# Autodesk Inventor assembly: Robot Assembly V1.5 - 6 wheel - toughbox mini - 24x28
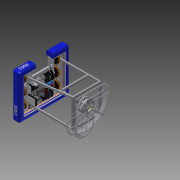
[picture p0: Inventor's stored thumbnail of the model, 180x180]
Saved by Autodesk Inventor 2013 (Build 170138000, 138)
## iProperties
Created: 2013-01-06
Part Number: Robot Assembly V1.5 - 6 wheel - toughbox mini - 24x28
Document SubType Name: Assembly
Designer: Moses
Mass: 19140.8 g
Surface Area: 65318.4 cm^2
Volume: 26385.5 cm^3
Density: 0.72543 g/cm^3
Author: Moses
## Documents named in this file (31)
- C:\Users\Moses\Documents\GitHub\frc2013CAD\Robot Assembly V1.5 - 6 wheel - toughbox mini - 24x28.iam
- C:\Users\Moses\Documents\GitHub\frc2013CAD\Drivetrain\Bearings\fr8zz-hex.ipt
- C:\Users\Moses\Documents\GitHub\frc2013CAD\Drivetrain\Drive Wheel Assembly V2.iam
- C:\Users\Moses\Documents\GitHub\frc2013CAD\Drivetrain\Standard Wheel Assembly V2.iam
- C:\Users\Moses\Documents\GitHub\frc2013CAD\Drivetrain\Toughbox-mini\Toughbox-mini-hex-long.iam
- C:\Users\Moses\Documents\GitHub\frc2013CAD\Drivetrain\6157K140 Shaft Collar\6157K140.ipt
- C:\Users\Moses\Documents\GitHub\frc2013CAD\Drivetrain\Shaft Spacer Part1.ipt
- C:\Users\Moses\Documents\GitHub\frc2013CAD\Drivetrain\Shaft Spacer Part2.ipt
- C:\Users\Moses\Documents\GitHub\frc2013CAD\Drivetrain\Shaft Spacer Part3.ipt
- C:\Users\Moses\Documents\GitHub\frc2013CAD\Drivetrain\Shaft Spacer Part4.ipt
- C:\Users\Moses\Documents\GitHub\frc2013CAD\Drivetrain\Shaft Spacer Part5.ipt
- C:\Users\Moses\Documents\GitHub\frc2013CAD\Drivetrain\Shaft Spacer Part6.ipt
- C:\Users\Moses\Documents\GitHub\frc2013CAD\Electrical\ELEC_Battery_NP18-12B.iam
- C:\Users\Moses\Documents\GitHub\frc2013CAD\Drivetrain\6061K130 Shaft\6061K130.ipt
- C:\Users\Moses\Documents\GitHub\frc2013CAD\Electrical\ELEC_CircuitBreaker_CB185-120.iam
- C:\Users\Moses\Documents\GitHub\frc2013CAD\Control Systems\CS_PowerBoard_A003206.ipt
- C:\Users\Moses\Documents\GitHub\frc2013CAD\Control Systems\CS_compactRIO_cRIO-FRC-II.ipt
- C:\Users\Moses\Documents\GitHub\frc2013CAD\Control Systems\CS_WirelessBridge_DAP1522.ipt
- C:\Users\Moses\Documents\GitHub\frc2013CAD\Control Systems\CS_Converter_CLL25-24S05.ipt
- C:\Users\Moses\Documents\GitHub\frc2013CAD\Control Systems\Talon.ipt
- C:\Users\Moses\Documents\GitHub\frc2013CAD\Drivetrain\Pneumatic_Compressor_VIAIR_00090\Pneumatic_Compressor_VIAIR_00090.iam
- C:\Users\Moses\Documents\GitHub\frc2013CAD\Drivetrain\Mounting Bracket V1.500 - (toughbox-mini - sheet metal).ipt
- C:\Users\Moses\Documents\GitHub\frc2013CAD\Drivetrain\Mounting Bracket V1.500 - (toughbox-mini - sheet metal - underside).ipt
- C:\Users\Moses\Documents\GitHub\frc2013CAD\Chassis\Chassis Assembly V1.500 24x28 Version.iam
- C:\Users\Moses\Documents\GitHub\frc2013CAD\Chassis\Bumpers\Bumper Assembly2 (24x28 robot).iam
- C:\Users\Moses\Documents\GitHub\frc2013CAD\Chassis\Bumpers\Bumper Assembly1 (24x28 robot).iam
- C:\Users\Moses\Documents\GitHub\frc2013CAD\Chassis\Bumpers\Bumper Assembly3 (24x28 robot).iam
- C:\Users\Moses\Documents\GitHub\frc2013CAD\Chassis\Bumpers\Bumper Assembly4 (24x28 robot).iam
- C:\Users\Moses\Documents\GitHub\frc2013CAD\Drivetrain\Bearing Block V1.500 Drivetrain.ipt
- C:\Users\Moses\Documents\GitHub\frc2013CAD\Drivetrain\Shaft Mount V1.500 Drivetrain.ipt
- C:\Users\Moses\Documents\GitHub\frc2013CAD\Launcher\Shooter\Shooter Assembly v2.iam
## Components (64 placed, 30 different names)
1. Chassis Assembly V1.500 24x28 Version:1 [sub-assembly] — Mate:1, Flush:1, Mate:2, Flush:4, Mate:3, Mate:4, Mate:5, Mate:8, Mate:9, Mate:10, Mate:17, Mate:18, Mate:19, Mate:20, Mate:21, Mate:26, Mate:27, Mate:28, Mate:29, Mate:34, Mate:35, Mate:36, Mate:37, Mate:42, Mate:43, Mate:44, Mate:47, Mate:48, Mate:51, Mate:52, Mate:55, Mate:83, Mate:84, Mate:85, Mate:89, Mate:98, Mate:99, Mate:100, Mate:101, Mate:115, Mate:116, Mate:117, Mate:118, Mate:119, Mate:120, Mate:125, Mate:126, Mate:127, Mate:128, Mate:129, Mate:130, Mate:132, Mate:136, Mate:141, Mate:142, Mate:143, Flush:16, Mate:144, Mate:145, Mate:146, Mate:147, Mate:148, Mate:149, Mate:150, Mate:151, Mate:152, Mate:153, Flush:17, Mate:154
2. Shooter Assembly v2:1 [sub-assembly] — Mate:153, Flush:17, Mate:154
3. Bumper Assembly1 (24x28 robot):1 [sub-assembly] — Mate:5, Mate:3, Flush:6, Flush:9, Flush:10
4. Bumper Assembly1 (24x28 robot):2 [sub-assembly] — Mate:1, Flush:1, Flush:3, Flush:2, Flush:7, Flush:8
5. Bumper Assembly2 (24x28 robot):1 [sub-assembly] — Mate:2, Flush:2, Flush:3, Flush:4, Mate:5, Flush:10
6. Bumper Assembly3 (24x28 robot):1 [sub-assembly] — Flush:9, Mate:5, Flush:6
7. Bumper Assembly4 (24x28 robot):1 [sub-assembly] — Mate:4, Flush:7, Flush:8
8. Pneumatic_Compressor_VIAIR_00090:1 [sub-assembly] — Mate:144
9. Shaft Spacer Part1:1 — Insert:111
10. Shaft Spacer Part2:1 — Insert:112
11. Shaft Spacer Part1:3 — Insert:113
12. Shaft Spacer Part2:2 — Insert:114
13. Shaft Spacer Part3:1 — Insert:115
14. Shaft Spacer Part3:2 — Insert:116
15. Shaft Spacer Part4:2 — Insert:117
16. Shaft Spacer Part4:1 — Insert:118
17. Shaft Spacer Part5:1 — Insert:119
18. Shaft Spacer Part5:2 — Insert:120
19. Shaft Spacer Part6:1 — Insert:121
20. Shaft Spacer Part6:2 — Insert:122
21. 6157K140:1 — Insert:107, Insert:113
22. 6157K140:2 — Insert:108, Insert:114
23. 6157K140:3 — Insert:110, Insert:111
24. 6157K140:4 — Insert:109, Insert:112
25. Toughbox-mini-hex-long:2 [sub-assembly] — Mate:131, Mate:132, Mate:133, Mate:134, Mate:135, Insert:118
26. Toughbox-mini-hex-long:1 [sub-assembly] — Mate:136, Mate:137, Mate:138, Mate:139, Mate:140, Insert:117
27. fr8zz-hex:1 — Insert:94, Insert:116
28. Bearing Block V1.500 Drivetrain:1 — Mate:83, Mate:84, Mate:85, Insert:106
29. Bearing Block V1.500 Drivetrain:2 — Mate:98, Mate:99, Mate:100, Insert:94
30. fr8zz-hex:2 — Insert:106, Insert:115
31. Mounting Bracket V1.500 - (toughbox-mini - sheet metal):1 — Mate:115, Mate:116, Mate:117, Mate:137, Mate:138
32. Mounting Bracket V1.500 - (toughbox-mini - sheet metal):2 — Mate:118, Mate:119, Mate:120, Mate:131, Mate:133
33. Mounting Bracket V1.500 - (toughbox-mini - sheet metal - underside):1 — Mate:125, Mate:126, Mate:127
34. Mounting Bracket V1.500 - (toughbox-mini - sheet metal - underside):2 — Mate:128, Mate:129, Mate:130
35. Shaft Mount V1.500 Drivetrain:8 — Mate:34, Mate:35, Mate:51, Insert:121
36. Shaft Mount V1.500 Drivetrain:7 — Mate:28, Mate:29, Mate:48, Insert:110
37. Shaft Mount V1.500 Drivetrain:6 — Mate:42, Mate:43, Mate:47, Insert:122
38. Shaft Mount V1.500 Drivetrain:5 — Mate:36, Mate:37, Mate:44, Insert:107
39. Shaft Mount V1.500 Drivetrain:4 — Mate:26, Mate:27, Mate:55, Insert:7, Insert:109
40. Shaft Mount V1.500 Drivetrain:3 — Mate:20, Mate:21, Mate:52, Insert:5, Insert:119
41. Shaft Mount V1.500 Drivetrain:2 — Mate:17, Mate:18, Mate:19, Insert:2, Insert:108
42. Shaft Mount V1.500 Drivetrain:1 — Mate:8, Mate:9, Mate:10, Insert:1, Insert:120
43. 6061K130:4 — Insert:7, Mate:21
44. 6061K130:3 — Insert:5, Mate:22
45. 6061K130:2 — Insert:2, Mate:19
46. 6061K130:1 — Insert:1, Mate:17
47. Standard Wheel Assembly V2:3 [sub-assembly] — Mate:17, Flush:13, Rotation:1
48. Drive Wheel Assembly V2:1 [sub-assembly] — Mate:89, Flush:13, Flush:15, Mate:139, Mate:140, Rotation:1, Rotation:2
49. Standard Wheel Assembly V2:1 [sub-assembly] — Mate:19, Flush:15, Rotation:2
50. Standard Wheel Assembly V2:2 [sub-assembly] — Mate:21, Flush:11, Rotation:4
51. Standard Wheel Assembly V2:4 [sub-assembly] — Mate:22, Flush:12, Rotation:3
52. Drive Wheel Assembly V2:2 [sub-assembly] — Mate:101, Flush:11, Flush:12, Mate:134, Mate:135, Rotation:3, Rotation:4
53. Talon:1 — Mate:147
54. Talon:2 — Mate:151
55. Talon:3 — Mate:146
56. Talon:4 — Mate:148
57. Talon:5 — Mate:149
58. Talon:6 — Mate:150
59. CS_Converter_CLL25-24S05:1 — Mate:145
60. CS_WirelessBridge_DAP1522:1 — Mate:152
61. CS_compactRIO_cRIO-FRC-II:1 — Flush:16
62. ELEC_CircuitBreaker_CB185-120:1 [sub-assembly] — Mate:142
63. ELEC_Battery_NP18-12B:1 [sub-assembly] — Mate:141
64. CS_PowerBoard_A003206:1 — Mate:143
## Relationships (119: Mate 78, Insert 22, Flush 15, RelateRotation 4)
- Mate:1: Chassis Assembly V1.500 24x28 Version:1 ↔ Bumper Assembly1 (24x28 robot):2
- Flush:1: Chassis Assembly V1.500 24x28 Version:1 ↔ Bumper Assembly1 (24x28 robot):2
- Mate:2: Chassis Assembly V1.500 24x28 Version:1 ↔ Bumper Assembly2 (24x28 robot):1
- Flush:2: Bumper Assembly1 (24x28 robot):2 ↔ Bumper Assembly2 (24x28 robot):1
- Flush:3: Bumper Assembly1 (24x28 robot):2 ↔ Bumper Assembly2 (24x28 robot):1
- Flush:4 (-69.85 mm): Chassis Assembly V1.500 24x28 Version:1 ↔ Bumper Assembly2 (24x28 robot):1
- Mate:5: Bumper Assembly1 (24x28 robot):1 ↔ Bumper Assembly2 (24x28 robot):1
- Mate:3: Chassis Assembly V1.500 24x28 Version:1 ↔ Bumper Assembly1 (24x28 robot):1
- Flush:6: Bumper Assembly1 (24x28 robot):1 ↔ Bumper Assembly3 (24x28 robot):1
- Mate:4: Chassis Assembly V1.500 24x28 Version:1 ↔ Bumper Assembly4 (24x28 robot):1
- Flush:7: Bumper Assembly1 (24x28 robot):2 ↔ Bumper Assembly4 (24x28 robot):1
- Flush:8: Bumper Assembly1 (24x28 robot):2 ↔ Bumper Assembly4 (24x28 robot):1
- Flush:9: Bumper Assembly1 (24x28 robot):1 ↔ Bumper Assembly3 (24x28 robot):1
- Flush:10: Bumper Assembly1 (24x28 robot):1 ↔ Bumper Assembly2 (24x28 robot):1
- Mate:5: Chassis Assembly V1.500 24x28 Version:1 ↔ Bumper Assembly3 (24x28 robot):1
- Insert:1 (-6.35 mm): Shaft Mount V1.500 Drivetrain:1 ↔ 6061K130:1
- Insert:2 (-6.35 mm): Shaft Mount V1.500 Drivetrain:2 ↔ 6061K130:2
- Insert:5 (-6.35 mm): Shaft Mount V1.500 Drivetrain:3 ↔ 6061K130:3
- Insert:7 (-6.35 mm): Shaft Mount V1.500 Drivetrain:4 ↔ 6061K130:4
- Mate:8: Chassis Assembly V1.500 24x28 Version:1 ↔ Shaft Mount V1.500 Drivetrain:1
- Mate:9: Chassis Assembly V1.500 24x28 Version:1 ↔ Shaft Mount V1.500 Drivetrain:1
- Mate:10: Chassis Assembly V1.500 24x28 Version:1 ↔ Shaft Mount V1.500 Drivetrain:1
- Mate:17: Chassis Assembly V1.500 24x28 Version:1 ↔ Shaft Mount V1.500 Drivetrain:2
- Mate:18: Chassis Assembly V1.500 24x28 Version:1 ↔ Shaft Mount V1.500 Drivetrain:2
- Mate:19: Chassis Assembly V1.500 24x28 Version:1 ↔ Shaft Mount V1.500 Drivetrain:2
- Mate:20: Chassis Assembly V1.500 24x28 Version:1 ↔ Shaft Mount V1.500 Drivetrain:3
- Mate:21: Chassis Assembly V1.500 24x28 Version:1 ↔ Shaft Mount V1.500 Drivetrain:3
- Mate:26: Chassis Assembly V1.500 24x28 Version:1 ↔ Shaft Mount V1.500 Drivetrain:4
- Mate:27: Chassis Assembly V1.500 24x28 Version:1 ↔ Shaft Mount V1.500 Drivetrain:4
- Mate:28: Chassis Assembly V1.500 24x28 Version:1 ↔ Shaft Mount V1.500 Drivetrain:7
- Mate:29: Chassis Assembly V1.500 24x28 Version:1 ↔ Shaft Mount V1.500 Drivetrain:7
- Mate:34: Chassis Assembly V1.500 24x28 Version:1 ↔ Shaft Mount V1.500 Drivetrain:8
- Mate:35: Chassis Assembly V1.500 24x28 Version:1 ↔ Shaft Mount V1.500 Drivetrain:8
- Mate:36: Chassis Assembly V1.500 24x28 Version:1 ↔ Shaft Mount V1.500 Drivetrain:5
- Mate:37: Chassis Assembly V1.500 24x28 Version:1 ↔ Shaft Mount V1.500 Drivetrain:5
- Mate:42: Chassis Assembly V1.500 24x28 Version:1 ↔ Shaft Mount V1.500 Drivetrain:6
- Mate:43: Chassis Assembly V1.500 24x28 Version:1 ↔ Shaft Mount V1.500 Drivetrain:6
- Mate:44: Chassis Assembly V1.500 24x28 Version:1 ↔ Shaft Mount V1.500 Drivetrain:5
- Mate:47: Chassis Assembly V1.500 24x28 Version:1 ↔ Shaft Mount V1.500 Drivetrain:6
- Mate:48: Chassis Assembly V1.500 24x28 Version:1 ↔ Shaft Mount V1.500 Drivetrain:7
- Mate:51: Chassis Assembly V1.500 24x28 Version:1 ↔ Shaft Mount V1.500 Drivetrain:8
- Mate:52: Chassis Assembly V1.500 24x28 Version:1 ↔ Shaft Mount V1.500 Drivetrain:3
- Mate:55: Chassis Assembly V1.500 24x28 Version:1 ↔ Shaft Mount V1.500 Drivetrain:4
- Mate:17: 6061K130:1 ↔ Standard Wheel Assembly V2:3
- Mate:19: 6061K130:2 ↔ Standard Wheel Assembly V2:1
- Mate:21: 6061K130:4 ↔ Standard Wheel Assembly V2:2
- Mate:22: 6061K130:3 ↔ Standard Wheel Assembly V2:4
- Mate:83: Chassis Assembly V1.500 24x28 Version:1 ↔ Bearing Block V1.500 Drivetrain:1
- Mate:84: Chassis Assembly V1.500 24x28 Version:1 ↔ Bearing Block V1.500 Drivetrain:1
- Mate:85: Chassis Assembly V1.500 24x28 Version:1 ↔ Bearing Block V1.500 Drivetrain:1
- Mate:89 (6.35 mm): Chassis Assembly V1.500 24x28 Version:1 ↔ Drive Wheel Assembly V2:1
- Insert:94: fr8zz-hex:1 ↔ Bearing Block V1.500 Drivetrain:2
- Mate:98: Chassis Assembly V1.500 24x28 Version:1 ↔ Bearing Block V1.500 Drivetrain:2
- Mate:99: Chassis Assembly V1.500 24x28 Version:1 ↔ Bearing Block V1.500 Drivetrain:2
- Mate:100: Chassis Assembly V1.500 24x28 Version:1 ↔ Bearing Block V1.500 Drivetrain:2
- Mate:101 (6.35 mm): Chassis Assembly V1.500 24x28 Version:1 ↔ Drive Wheel Assembly V2:2
- Insert:106: Bearing Block V1.500 Drivetrain:1 ↔ fr8zz-hex:2
- Mate:115: Chassis Assembly V1.500 24x28 Version:1 ↔ Mounting Bracket V1.500 - (toughbox-mini - sheet metal):1
- Mate:116: Chassis Assembly V1.500 24x28 Version:1 ↔ Mounting Bracket V1.500 - (toughbox-mini - sheet metal):1
- Mate:117: Chassis Assembly V1.500 24x28 Version:1 ↔ Mounting Bracket V1.500 - (toughbox-mini - sheet metal):1
- Mate:118: Chassis Assembly V1.500 24x28 Version:1 ↔ Mounting Bracket V1.500 - (toughbox-mini - sheet metal):2
- Mate:119: Chassis Assembly V1.500 24x28 Version:1 ↔ Mounting Bracket V1.500 - (toughbox-mini - sheet metal):2
- Mate:120: Chassis Assembly V1.500 24x28 Version:1 ↔ Mounting Bracket V1.500 - (toughbox-mini - sheet metal):2
- Flush:11: Standard Wheel Assembly V2:2 ↔ Drive Wheel Assembly V2:2
- Flush:12: Standard Wheel Assembly V2:4 ↔ Drive Wheel Assembly V2:2
- Flush:13: Standard Wheel Assembly V2:3 ↔ Drive Wheel Assembly V2:1
- Mate:125: Chassis Assembly V1.500 24x28 Version:1 ↔ Mounting Bracket V1.500 - (toughbox-mini - sheet metal - underside):1
- Mate:126: Chassis Assembly V1.500 24x28 Version:1 ↔ Mounting Bracket V1.500 - (toughbox-mini - sheet metal - underside):1
- Mate:127: Chassis Assembly V1.500 24x28 Version:1 ↔ Mounting Bracket V1.500 - (toughbox-mini - sheet metal - underside):1
- Mate:128: Chassis Assembly V1.500 24x28 Version:1 ↔ Mounting Bracket V1.500 - (toughbox-mini - sheet metal - underside):2
- Mate:129: Chassis Assembly V1.500 24x28 Version:1 ↔ Mounting Bracket V1.500 - (toughbox-mini - sheet metal - underside):2
- Mate:130: Chassis Assembly V1.500 24x28 Version:1 ↔ Mounting Bracket V1.500 - (toughbox-mini - sheet metal - underside):2
- Flush:15: Drive Wheel Assembly V2:1 ↔ Standard Wheel Assembly V2:1
- Mate:131: Toughbox-mini-hex-long:2 ↔ Mounting Bracket V1.500 - (toughbox-mini - sheet metal):2
- Mate:132: Chassis Assembly V1.500 24x28 Version:1 ↔ Toughbox-mini-hex-long:2
- Mate:133: Toughbox-mini-hex-long:2 ↔ Mounting Bracket V1.500 - (toughbox-mini - sheet metal):2
- Mate:134: Toughbox-mini-hex-long:2 ↔ Drive Wheel Assembly V2:2
- Mate:135: Toughbox-mini-hex-long:2 ↔ Drive Wheel Assembly V2:2
- Mate:136: Chassis Assembly V1.500 24x28 Version:1 ↔ Toughbox-mini-hex-long:1
- Mate:137: Toughbox-mini-hex-long:1 ↔ Mounting Bracket V1.500 - (toughbox-mini - sheet metal):1
- Mate:138: Toughbox-mini-hex-long:1 ↔ Mounting Bracket V1.500 - (toughbox-mini - sheet metal):1
- Mate:139: Toughbox-mini-hex-long:1 ↔ Drive Wheel Assembly V2:1
- Mate:140: Toughbox-mini-hex-long:1 ↔ Drive Wheel Assembly V2:1
- Rotation:1 [RelateRotation] (1 ul): Standard Wheel Assembly V2:3 ↔ Drive Wheel Assembly V2:1
- Rotation:2 [RelateRotation] (1 ul): Drive Wheel Assembly V2:1 ↔ Standard Wheel Assembly V2:1
- Rotation:3 [RelateRotation] (1 ul): Standard Wheel Assembly V2:4 ↔ Drive Wheel Assembly V2:2
- Rotation:4 [RelateRotation] (1 ul): Standard Wheel Assembly V2:2 ↔ Drive Wheel Assembly V2:2
- Insert:107: 6157K140:1 ↔ Shaft Mount V1.500 Drivetrain:5
- Insert:108: 6157K140:2 ↔ Shaft Mount V1.500 Drivetrain:2
- Insert:109: 6157K140:4 ↔ Shaft Mount V1.500 Drivetrain:4
- Insert:110: 6157K140:3 ↔ Shaft Mount V1.500 Drivetrain:7
- Insert:111: Shaft Spacer Part1:1 ↔ 6157K140:3
- Insert:112: Shaft Spacer Part2:1 ↔ 6157K140:4
- Insert:113: Shaft Spacer Part1:3 ↔ 6157K140:1
- Insert:114: Shaft Spacer Part2:2 ↔ 6157K140:2
- Insert:115: Shaft Spacer Part3:1 ↔ fr8zz-hex:2
- Insert:116: Shaft Spacer Part3:2 ↔ fr8zz-hex:1
- Insert:117: Shaft Spacer Part4:2 ↔ Toughbox-mini-hex-long:1
- Insert:118: Shaft Spacer Part4:1 ↔ Toughbox-mini-hex-long:2
- Insert:119: Shaft Spacer Part5:1 ↔ Shaft Mount V1.500 Drivetrain:3
- Insert:120: Shaft Spacer Part5:2 ↔ Shaft Mount V1.500 Drivetrain:1
- Insert:121: Shaft Spacer Part6:1 ↔ Shaft Mount V1.500 Drivetrain:8
- Insert:122: Shaft Spacer Part6:2 ↔ Shaft Mount V1.500 Drivetrain:6
- Mate:141: Chassis Assembly V1.500 24x28 Version:1 ↔ ELEC_Battery_NP18-12B:1
- Mate:142: Chassis Assembly V1.500 24x28 Version:1 ↔ ELEC_CircuitBreaker_CB185-120:1
- Mate:143: Chassis Assembly V1.500 24x28 Version:1 ↔ CS_PowerBoard_A003206:1
- Flush:16: Chassis Assembly V1.500 24x28 Version:1 ↔ CS_compactRIO_cRIO-FRC-II:1
- Mate:144: Chassis Assembly V1.500 24x28 Version:1 ↔ Pneumatic_Compressor_VIAIR_00090:1
- Mate:145: Chassis Assembly V1.500 24x28 Version:1 ↔ CS_Converter_CLL25-24S05:1
- Mate:146: Chassis Assembly V1.500 24x28 Version:1 ↔ Talon:3
- Mate:147: Chassis Assembly V1.500 24x28 Version:1 ↔ Talon:1
- Mate:148: Chassis Assembly V1.500 24x28 Version:1 ↔ Talon:4
- Mate:149: Chassis Assembly V1.500 24x28 Version:1 ↔ Talon:5
- Mate:150: Chassis Assembly V1.500 24x28 Version:1 ↔ Talon:6
- Mate:151: Chassis Assembly V1.500 24x28 Version:1 ↔ Talon:2
- Mate:152: Chassis Assembly V1.500 24x28 Version:1 ↔ CS_WirelessBridge_DAP1522:1
- Mate:153: Chassis Assembly V1.500 24x28 Version:1 ↔ Shooter Assembly v2:1
- Flush:17: Chassis Assembly V1.500 24x28 Version:1 ↔ Shooter Assembly v2:1
- Mate:154: Chassis Assembly V1.500 24x28 Version:1 ↔ Shooter Assembly v2:1
